# Autodesk Inventor assembly: RasPi_Camera
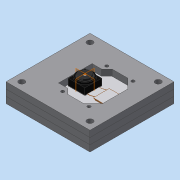
[picture p0: Inventor's stored thumbnail of the model, 180x180]
Saved by Autodesk Inventor 2016 SP1 (Build 200210100, 210)
## iProperties
Created: 2013-09-06
Part Number: RasPi_Camera
Document SubType Name: Assembly
Designer: Mohamed A.
Sending System: SolidWorks 2014
Last Author: lavirott
Last Saved: 2016-01-23
Author: DFKI GmbH
Comments: http://www.dfki.de/robotik
## Documents named in this file (5)
- C:\Users\Mohamed\Documents\inventor\StemCellsPlatform\Camera\Raspberry Pi Camera rev 1.3\RasPi_Camera.iam
- C:\Users\Mohamed\Documents\inventor\StemCellsPlatform\Camera\Raspberry Pi Camera rev 1.3\RasPi_Camera_Board.ipt
- C:\Users\Mohamed\Documents\inventor\StemCellsPlatform\Camera\Raspberry Pi Camera rev 1.3\OVA5647.iam
- C:\Users\Mohamed\Documents\inventor\StemCellsPlatform\Laser Cut\Camera-Holder\Camera-Holder_Mount.ipt
- C:\Users\Mohamed\Documents\inventor\StemCellsPlatform\Laser Cut\Camera-Holder\Camera-Holder_Mount-Bottom.ipt
## Components (5 placed, 4 different names)
1. RasPi_Camera_Board:1 — Mate:1, Insert:1, Insert:2
2. OVA5647:2 [sub-assembly]
3. Camera-Holder_Mount:1 — Mate:1, Insert:1, Insert:2, Flush:1
4. Camera-Holder_Mount-Bottom:1 — Flush:1, Mate:2, Insert:3, Insert:4
5. Camera-Holder_Mount-Bottom:2 — Mate:2, Insert:3, Insert:4
## Relationships (7: Insert 4, Mate 2, Flush 1)
- Mate:1: RasPi_Camera_Board:1 ↔ Camera-Holder_Mount:1
- Insert:1: RasPi_Camera_Board:1 ↔ Camera-Holder_Mount:1
- Insert:2: RasPi_Camera_Board:1 ↔ Camera-Holder_Mount:1
- Flush:1: Camera-Holder_Mount:1 ↔ Camera-Holder_Mount-Bottom:1
- Mate:2: Camera-Holder_Mount-Bottom:1 ↔ Camera-Holder_Mount-Bottom:2
- Insert:3: Camera-Holder_Mount-Bottom:1 ↔ Camera-Holder_Mount-Bottom:2
- Insert:4: Camera-Holder_Mount-Bottom:1 ↔ Camera-Holder_Mount-Bottom:2
